# Autodesk Inventor assembly: DonjaKonstrukcija_v.5.0.
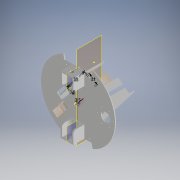
[picture p0: Inventor's stored thumbnail of the model, 180x180]
Saved by Autodesk Inventor 2020 (Build 240168000, 168)
## iProperties
Created: 2020-12-12
Part Number: DonjaKonstrukcija_v.5.0.
Document SubType Name: Assembly
Designer: Sičaja
Author: Sičaja
## Documents named in this file (4)
- C:\Users\Sicaja\Documents\Projects\3D Drawings\Inventor_draws\Robocup\Inverntor_parts_for_print\1_NewScratches\DonjaKonstrukcija_v.5.0..iam
- C:\Users\Sicaja\Documents\Projects\3D Drawings\Inventor_draws\Robocup\Inverntor_parts_for_print\1_NewScratches\DonjaKonstrukcija_v.5.0.ipt
- C:\Users\Sicaja\Documents\Projects\3D Drawings\Inventor_draws\Robocup\Inverntor_parts_for_print\DrzacZaMotor.ipt
- C:\Users\Sicaja\Documents\Projects\3D Drawings\Inventor_draws\Robocup\Inverntor_parts_for_print\DropMechanism_v.2.0.ipt
## Components (4 placed, 3 different names)
1. DonjaKonstrukcija_v.5.0:1 — Mate:1, Flush:1, Flush:2, Mate:3, Flush:4, Mate:5, Mate:6, Flush:6
2. DrzacZaMotor:1 — Mate:1, Flush:2, Flush:3
3. DrzacZaMotor:2 — Mate:3, Flush:4, Flush:5
4. DropMechanism_v.2.0:1 — Mate:5, Mate:6, Flush:6
## Relationships (12: Mate 6, Flush 6)
- Mate:1: DonjaKonstrukcija_v.5.0:1 ↔ DrzacZaMotor:1
- Flush:1 (-1 mm): DonjaKonstrukcija_v.5.0:1
- Flush:2: DonjaKonstrukcija_v.5.0:1 ↔ DrzacZaMotor:1
- Flush:3 (-13 mm): DrzacZaMotor:1
- Mate:2
- Mate:3: DonjaKonstrukcija_v.5.0:1 ↔ DrzacZaMotor:2
- Flush:4: DonjaKonstrukcija_v.5.0:1 ↔ DrzacZaMotor:2
- Flush:5 (-13 mm): DrzacZaMotor:2
- Mate:4
- Mate:5: DonjaKonstrukcija_v.5.0:1 ↔ DropMechanism_v.2.0:1
- Mate:6: DonjaKonstrukcija_v.5.0:1 ↔ DropMechanism_v.2.0:1
- Flush:6: DonjaKonstrukcija_v.5.0:1 ↔ DropMechanism_v.2.0:1
